# Autodesk Inventor assembly: Boat_Bot_Assembly
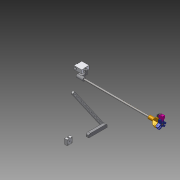
[picture p0: Inventor's stored thumbnail of the model, 180x180]
Saved by Autodesk Inventor 2014 SP1 (Build 180222100, 222)
## iProperties
Created: 2014-01-22
Part Number: Boat_Bot_Assembly
Document SubType Name: Assembly
Designer: tom
Author: tom
## Documents named in this file (9)
- C:\Users\tom\Documents\GitHub\Boat_Bot\Inventor\Boat_Bot_Assembly.iam
- C:\Users\tom\Documents\GitHub\Belt_Cutter\Beam2.ipt
- C:\Users\tom\Documents\GitHub\Boat_Bot\Inventor\Arm Tube.ipt
- C:\Users\tom\Documents\GitHub\Boat_Bot\Inventor\Base.ipt
- C:\Users\tom\Documents\GitHub\Boat_Bot\Inventor\Channel Bracket B.ipt
- C:\Users\tom\Documents\GitHub\Boat_Bot\Inventor\Tube Bracket.ipt
- C:\Users\tom\Documents\GitHub\Boat_Bot\Inventor\Claw.iam
- C:\Users\tom\Documents\GitHub\Delta_Robots\Delatabot - Small Model\Inventor\Deltabot - Small Model\Component2.ipt
- C:\Users\tom\Documents\GitHub\Boat_Bot\Inventor\Servo Bracket.ipt
## Components (8 placed, 8 different names)
1. Base:1 — Mate:1, Rotational:1
2. Arm Tube:1 — Mate:6
3. Beam2:1 — Rotational:1
4. Channel Bracket B:1
5. Tube Bracket:1
6. Claw:1 [sub-assembly]
7. Servo — Mate:3, Mate:4, Mate:5
8. Servo Bracket:1 — Mate:3, Mate:4, Mate:5, Mate:6
## Relationships (7: Mate 6, RevoluteJoint 1)
- Mate:1: Base:1
- Rotational:1 [RevoluteJoint]: Base:1 ↔ Beam2:1
- [Mate]: Arm Tube:1 ↔ Claw:1
- Mate:3: Servo ↔ Servo Bracket:1
- Mate:4 (1 mm): Servo ↔ Servo Bracket:1
- Mate:5 (1 mm): Servo ↔ Servo Bracket:1
- Mate:6: Arm Tube:1 ↔ Servo Bracket:1
